# Autodesk Inventor assembly: Motor assembly
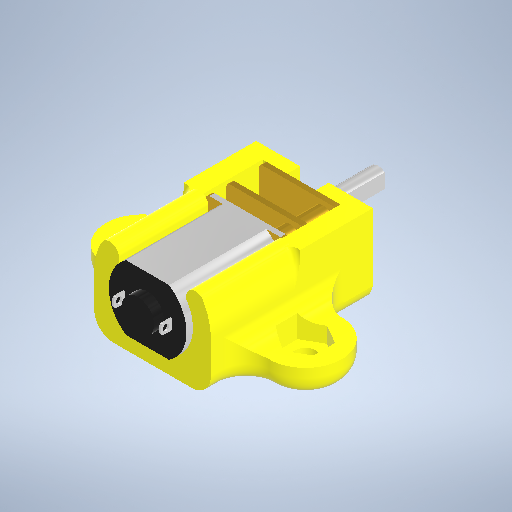
[picture p0: Inventor's stored thumbnail of the model, 512x512]
Saved by Autodesk Inventor 2025.1 (Build 291241000, 241)
## iProperties
Created: 2024-10-03
Part Number: Motor assembly
Document SubType Name: Assembly
Designer: bw1293
Author: bw1293
## Documents named in this file (4)
- C:\0_RDAC\Bw RDAC 1\Motor assembly.iam
- C:\0_RDAC\Bw RDAC 1\wheel.ipt
- C:\0_RDAC\Bw RDAC 1\MotorHolder.ipt
- C:\0_RDAC\Bw RDAC 1\Pololu_MMG_Motor.ipt
## Components (3 placed, 3 different names)
1. wheel:1 — Insert:1
2. MotorHolder:1 — Mate:1, Mate:2, Mate:3
3. Pololu_MMG_Motor:1 — Mate:1, Mate:2, Mate:3, Insert:1
## Relationships (4: Mate 3, Insert 1)
- Mate:1: MotorHolder:1 ↔ Pololu_MMG_Motor:1
- Mate:2: MotorHolder:1 ↔ Pololu_MMG_Motor:1
- Mate:3: MotorHolder:1 ↔ Pololu_MMG_Motor:1
- Insert:1 (-8 mm): wheel:1 ↔ Pololu_MMG_Motor:1
